# Autodesk Inventor assembly: fc18-084
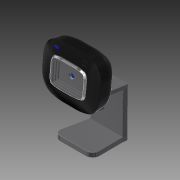
[picture p0: Inventor's stored thumbnail of the model, 180x180]
Saved by Autodesk Inventor 2018 (Build 220112000, 112)
## iProperties
Category: Electronics
Company: Autodesk Inc.
Created: 2017-11-27
Part Number: fc18-084
Document SubType Name: Assembly
Designer: Autodesk Inc.
Catalog Web Link: http://www.microsoft.com/accessories/en-us/products/webcams/lifecam-hd-3000/t3h-00011#details
Vendor: Microsoft Inc.
Author: Autodesk Inc.
Keywords: FIRSTChoice
## Documents named in this file (3)
- F:\FIRST 2018\FIRST 2018 FirstChoice\fc18-084_Camera.iam
- F:\FIRST 2018\FIRST 2018 FirstChoice\Parts\CS_Camera_HD3000.ipt
- F:\FIRST 2018\FIRST 2018 FirstChoice\Parts\CS_Camera_HD3000_Base_01.ipt
## Components (2 placed, 2 different names)
1. CS_Camera_HD3000:1 — Mate:1, Mate:2
2. CS_Camera_HD3000_Base_01:1 — Mate:1, Mate:2
## Relationships (2: Mate 2)
- Mate:1: CS_Camera_HD3000:1 ↔ CS_Camera_HD3000_Base_01:1
- Mate:2: CS_Camera_HD3000:1 ↔ CS_Camera_HD3000_Base_01:1
